# Autodesk Inventor assembly: CNC_lower_skirt
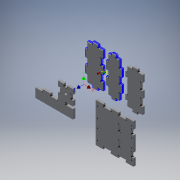
[picture p0: Inventor's stored thumbnail of the model, 180x180]
Saved by Autodesk Inventor 2016 SP2 (Build 200236200, 236)
## iProperties
Created: 2017-09-11
Part Number: CNC_lower_skirt
Document SubType Name: Assembly
Designer: Admin
Author: Admin
## Documents named in this file (6)
- E:\DATA\Inventor\AtongJali_v2\CNC_lower_skirt.iam
- E:\DATA\Inventor\AtongJali_v2\base_plate_1.ipt
- E:\DATA\Inventor\AtongJali_v2\step_mount_center_1.ipt
- E:\DATA\Inventor\AtongJali_v2\step_mount_front_1.ipt
- E:\DATA\Inventor\AtongJali_v2\step_mount_top_1.ipt
- E:\DATA\Inventor\AtongJali_v2\stepper_mount_L_1.ipt
## Components (5 placed, 5 different names)
1. base_plate_1:1 — Flush:4, Flush:5
2. step_mount_center_1:1 — Flush:3, Flush:4
3. step_mount_front_1:1 — Flush:2, Flush:3
4. step_mount_top_1:1 — Flush:2
5. stepper_mount_L_1:1 — Flush:5
## Relationships (4: Flush 4)
- Flush:2: step_mount_front_1:1 ↔ step_mount_top_1:1
- Flush:3: step_mount_center_1:1 ↔ step_mount_front_1:1
- Flush:4: base_plate_1:1 ↔ step_mount_center_1:1
- Flush:5: base_plate_1:1 ↔ stepper_mount_L_1:1
